# Autodesk Inventor assembly: Ring, Sub Assembly
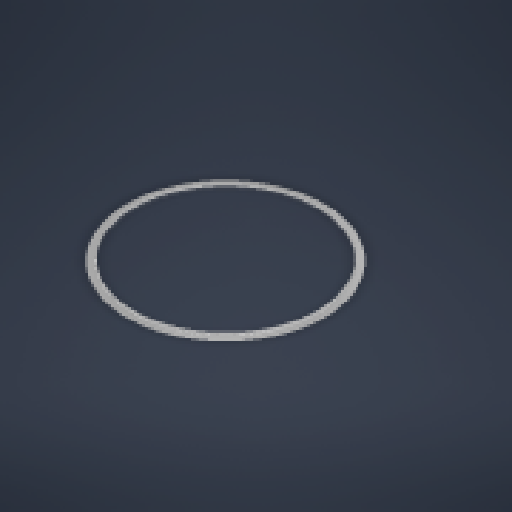
[picture p0: Inventor's stored thumbnail of the model, 512x512]
Saved by Autodesk Inventor 2026 (Build 300175000, 175)
## iProperties
Created: 2025-11-03
Part Number: Ring, Sub Assembly
Document SubType Name: Assembly
Designer: Brandon Portillo
Mass: 43763.3 g
Surface Area: 54614.1 cm^2
Volume: 16208.6 cm^3
Density: 2.7 g/cm^3
Author: Brandon Portillo
## Documents named in this file (2)
- C:\Users\anarc\GitHub\TSGC-NASA_Senior_Design\CAD\Pressure Vessel\Ring, Sub Assembly.iam
- C:\Users\anarc\GitHub\TSGC-NASA_Senior_Design\CAD\Pressure Vessel\Support Ring Section, L Section.ipt
## Components (3 placed, 1 different names)
1. Support Ring Section, L Section:1 — Mate:1, Flush:1, Mate:2
2. Support Ring Section, L Section:2 — Mate:1, Flush:1, Mate:2, Mate:3, Mate:4, Flush:2
3. Support Ring Section, L Section:3 — Mate:3, Mate:4, Flush:2
## Relationships (6: Mate 4, Flush 2)
- Mate:1: Support Ring Section, L Section:1 ↔ Support Ring Section, L Section:2
- Flush:1: Support Ring Section, L Section:1 ↔ Support Ring Section, L Section:2
- Mate:2: Support Ring Section, L Section:1 ↔ Support Ring Section, L Section:2
- Mate:3: Support Ring Section, L Section:2 ↔ Support Ring Section, L Section:3
- Mate:4: Support Ring Section, L Section:2 ↔ Support Ring Section, L Section:3
- Flush:2: Support Ring Section, L Section:2 ↔ Support Ring Section, L Section:3
